# Autodesk Inventor assembly: Drivetrain Side
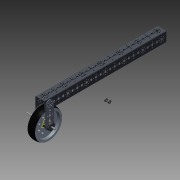
[picture p0: Inventor's stored thumbnail of the model, 180x180]
Saved by Autodesk Inventor 2015 (Build 190159000, 159)
## iProperties
Created: 2015-09-28
Part Number: Drivetrain Side
Document SubType Name: Assembly
Designer: Jing-Chen
Author: Jing-Chen
## Documents named in this file (8)
- C:\Users\Jing-Chen\Desktop\Bionic Hybrids 2016\Bionic-Hybrids\CAD\Drivetrain\Sub-Assemblies\Drivetrain Side.iam
- C:\Users\Jing-Chen\Desktop\Bionic Hybrids 2016\Bionic-Hybrids\Stock\Bracket-U25 - 739069.ipt
- C:\Users\Jing-Chen\Desktop\Bionic Hybrids 2016\Bionic-Hybrids\Stock\Plate-5x1 - 739273.ipt
- C:\Users\Jing-Chen\Desktop\Bionic Hybrids 2016\Bionic-Hybrids\CAD\Drivetrain\Sub-Assemblies\Wheel Assembly.iam
- C:\Users\Jing-Chen\Desktop\Bionic Hybrids 2016\Bionic-Hybrids\Stock\Spacer 3.125mm- 739100.ipt
- C:\Users\Jing-Chen\Desktop\Bionic Hybrids 2016\Bionic-Hybrids\Stock\Axle-100mm - 739088.ipt
- C:\Users\Jing-Chen\Desktop\Bionic Hybrids 2016\Bionic-Hybrids\CAD\Drivetrain\Modified Parts\Axle Hub - non-locking.ipt
- C:\Users\Jing-Chen\Desktop\Bionic Hybrids 2016\Bionic-Hybrids\Stock\Screw 7.938mm - 739098.ipt
## Components (14 placed, 7 different names)
1. Bracket-U25 - 739069:1 — Mate:1, Mate:2, Mate:3, Mate:4, Mate:5, Mate:6
2. Plate-5x1 - 739273:1 — Mate:1, Mate:2, Mate:3, Mate:7, Mate:14
3. Plate-5x1 - 739273:2 — Mate:4, Mate:5, Mate:6, Mate:16, Mate:18, Mate:19, Mate:20, Mate:21, Mate:22, Mate:23, Mate:24, Mate:25, Mate:26
4. Wheel Assembly:1 [sub-assembly] — Mate:8, Mate:29
5. Spacer 3.125mm- 739100:1
6. Spacer 3.125mm- 739100:2
7. Spacer 3.125mm- 739100:3 — Mate:27, Mate:28, Mate:29
8. Axle-100mm - 739088:1 — Mate:7, Mate:8, Mate:13, Mate:15, Mate:27
9. Axle Hub - non-locking:1 — Mate:15, Mate:16, Mate:18
10. Axle Hub - non-locking:2 — Mate:13, Mate:14, Mate:28
11. Screw 7.938mm - 739098:1 — Mate:19, Mate:20
12. Screw 7.938mm - 739098:2 — Mate:23, Mate:26
13. Screw 7.938mm - 739098:3 — Mate:24, Mate:25
14. Screw 7.938mm - 739098:4 — Mate:21, Mate:22
## Relationships (24: Mate 24)
- Mate:1: Bracket-U25 - 739069:1 ↔ Plate-5x1 - 739273:1
- Mate:2: Bracket-U25 - 739069:1 ↔ Plate-5x1 - 739273:1
- Mate:3: Bracket-U25 - 739069:1 ↔ Plate-5x1 - 739273:1
- Mate:4: Bracket-U25 - 739069:1 ↔ Plate-5x1 - 739273:2
- Mate:5: Bracket-U25 - 739069:1 ↔ Plate-5x1 - 739273:2
- Mate:6: Bracket-U25 - 739069:1 ↔ Plate-5x1 - 739273:2
- Mate:7: Plate-5x1 - 739273:1 ↔ Axle-100mm - 739088:1
- Mate:8: Wheel Assembly:1 ↔ Axle-100mm - 739088:1
- Mate:13: Axle-100mm - 739088:1 ↔ Axle Hub - non-locking:2
- Mate:14: Plate-5x1 - 739273:1 ↔ Axle Hub - non-locking:2
- Mate:15: Axle-100mm - 739088:1 ↔ Axle Hub - non-locking:1
- Mate:16: Plate-5x1 - 739273:2 ↔ Axle Hub - non-locking:1
- Mate:18: Plate-5x1 - 739273:2 ↔ Axle Hub - non-locking:1
- Mate:19: Plate-5x1 - 739273:2 ↔ Screw 7.938mm - 739098:1
- Mate:20: Plate-5x1 - 739273:2 ↔ Screw 7.938mm - 739098:1
- Mate:21: Plate-5x1 - 739273:2 ↔ Screw 7.938mm - 739098:4
- Mate:22: Plate-5x1 - 739273:2 ↔ Screw 7.938mm - 739098:4
- Mate:23: Plate-5x1 - 739273:2 ↔ Screw 7.938mm - 739098:2
- Mate:24: Plate-5x1 - 739273:2 ↔ Screw 7.938mm - 739098:3
- Mate:25: Plate-5x1 - 739273:2 ↔ Screw 7.938mm - 739098:3
- Mate:26: Plate-5x1 - 739273:2 ↔ Screw 7.938mm - 739098:2
- Mate:27: Spacer 3.125mm- 739100:3 ↔ Axle-100mm - 739088:1
- Mate:28: Spacer 3.125mm- 739100:3 ↔ Axle Hub - non-locking:2
- Mate:29: Wheel Assembly:1 ↔ Spacer 3.125mm- 739100:3
